# Autodesk Inventor assembly: B_Legs0_MIR
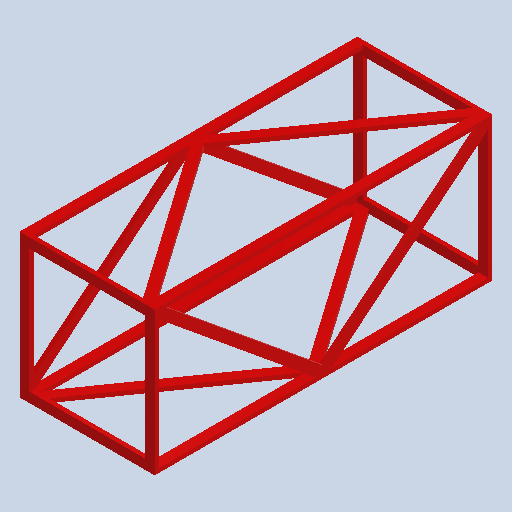
[picture p0: Inventor's stored thumbnail of the model, 512x512]
Saved by Autodesk Inventor 2025 (Build 290162000, 162)
## iProperties
Created: 2024-09-19
Part Number: B_Legs0_MIR
Document SubType Name: Assembly
Designer: localadmin
Author: User
## Documents named in this file (6)
- C:\Users\localadmin\Documents\USCTigerBurn24\Tburn24\F_Legs1\B_Legs0_MIR.iam
- C:\Users\localadmin\Documents\USCTigerBurn24\Tburn24\F_Legs1\8'x2x4_MIR.ipt
- C:\Users\localadmin\Documents\USCTigerBurn24\Tburn24\F_Legs1\4x2x4_MIR.ipt
- C:\Users\localadmin\Documents\USCTigerBurn24\Tburn24\F_Legs1\3'5x2x4_MIR.ipt
- C:\Users\localadmin\Documents\USCTigerBurn24\Tburn24\F_Legs1\side1_MIR.ipt
- C:\Users\localadmin\Documents\USCTigerBurn24\Tburn24\F_Legs1\side2_MIR.ipt
## Components (16 placed, 5 different names)
1. 8'x2x4_MIR:1 — Flush:3, Flush:2, Flush:1, Flush:14, Flush:13, Flush:8, Flush:12, Flush:10, Mate:3, Flush:22
2. 8'x2x4_MIR:2 — Flush:3, Flush:2, Flush:1, Mate:1, Flush:16, Flush:15, Mate:5, Flush:11, Flush:9, Flush:27, Flush:31, Mate:19, Flush:32, Mate:21
3. 4x2x4_MIR:1 — Flush:14, Flush:13, Flush:8, Mate:14, Flush:20, Flush:17, Mate:7, Flush:21, Mate:15, Flush:23, Mate:16, Flush:29
4. 4x2x4_MIR:2 — Flush:16, Flush:15, Mate:5, Flush:19, Flush:18, Mate:6, Mate:22
5. 4x2x4_MIR:3 — Flush:11, Flush:9, Flush:25, Flush:26
6. 4x2x4_MIR:4 — Flush:12, Flush:10, Mate:3, Mate:18, Mate:17
7. 8'x2x4_MIR:3 — Mate:14, Flush:20, Flush:17, Mate:7, Flush:24, Flush:30
8. 8'x2x4_MIR:4 — Flush:19, Flush:18, Mate:6, Flush:28
9. 3'5x2x4_MIR:1 — Flush:22, Flush:21, Mate:15
10. 3'5x2x4_MIR:2 — Flush:24, Flush:23, Mate:16
11. 3'5x2x4_MIR:3 — Flush:28, Flush:25, Mate:18
12. 3'5x2x4_MIR:4 — Flush:27, Flush:26, Mate:17, Mate:20
13. side1_MIR:1 — Flush:29
14. side2_MIR:1 — Flush:30
15. side2_MIR:2 — Flush:31, Mate:20, Mate:19
16. side1_MIR:2 — Flush:32, Mate:22, Mate:21
## Relationships (42: Flush 25, Mate 17)
- Flush:3: 8'x2x4_MIR:1 ↔ 8'x2x4_MIR:2
- Flush:2 (1130.3 mm): 8'x2x4_MIR:1 ↔ 8'x2x4_MIR:2
- Flush:1: 8'x2x4_MIR:1 ↔ 8'x2x4_MIR:2
- Mate:1: 8'x2x4_MIR:2
- Flush:14: 8'x2x4_MIR:1 ↔ 4x2x4_MIR:1
- Flush:13: 8'x2x4_MIR:1 ↔ 4x2x4_MIR:1
- Flush:8 [Mate]: 8'x2x4_MIR:1 ↔ 4x2x4_MIR:1
- Flush:16: 8'x2x4_MIR:2 ↔ 4x2x4_MIR:2
- Flush:15: 8'x2x4_MIR:2 ↔ 4x2x4_MIR:2
- Mate:5: 8'x2x4_MIR:2 ↔ 4x2x4_MIR:2
- Flush:11: 8'x2x4_MIR:2 ↔ 4x2x4_MIR:3
- Flush:9: 8'x2x4_MIR:2 ↔ 4x2x4_MIR:3
- Flush:12: 8'x2x4_MIR:1 ↔ 4x2x4_MIR:4
- Flush:10: 8'x2x4_MIR:1 ↔ 4x2x4_MIR:4
- Mate:3: 8'x2x4_MIR:1 ↔ 4x2x4_MIR:4
- Mate:14: 4x2x4_MIR:1 ↔ 8'x2x4_MIR:3
- Flush:20: 4x2x4_MIR:1 ↔ 8'x2x4_MIR:3
- Flush:17: 4x2x4_MIR:1 ↔ 8'x2x4_MIR:3
- Mate:7: 4x2x4_MIR:1 ↔ 8'x2x4_MIR:3
- Flush:19: 4x2x4_MIR:2 ↔ 8'x2x4_MIR:4
- Flush:18: 4x2x4_MIR:2 ↔ 8'x2x4_MIR:4
- Mate:6: 4x2x4_MIR:2 ↔ 8'x2x4_MIR:4
- Flush:22: 8'x2x4_MIR:1 ↔ 3'5x2x4_MIR:1
- Flush:21: 4x2x4_MIR:1 ↔ 3'5x2x4_MIR:1
- Mate:15: 4x2x4_MIR:1 ↔ 3'5x2x4_MIR:1
- Flush:24: 8'x2x4_MIR:3 ↔ 3'5x2x4_MIR:2
- Flush:23: 4x2x4_MIR:1 ↔ 3'5x2x4_MIR:2
- Mate:16: 4x2x4_MIR:1 ↔ 3'5x2x4_MIR:2
- Flush:28: 8'x2x4_MIR:4 ↔ 3'5x2x4_MIR:3
- Flush:25: 4x2x4_MIR:3 ↔ 3'5x2x4_MIR:3
- Mate:18: 4x2x4_MIR:4 ↔ 3'5x2x4_MIR:3
- Flush:27: 8'x2x4_MIR:2 ↔ 3'5x2x4_MIR:4
- Flush:26: 4x2x4_MIR:3 ↔ 3'5x2x4_MIR:4
- Mate:17: 4x2x4_MIR:4 ↔ 3'5x2x4_MIR:4
- Flush:29 [Mate]: 4x2x4_MIR:1 ↔ side1_MIR:1
- Flush:30 [Mate]: 8'x2x4_MIR:3 ↔ side2_MIR:1
- Flush:31: 8'x2x4_MIR:2 ↔ side2_MIR:2
- Mate:20: 3'5x2x4_MIR:4 ↔ side2_MIR:2
- Mate:19: 8'x2x4_MIR:2 ↔ side2_MIR:2
- Flush:32: 8'x2x4_MIR:2 ↔ side1_MIR:2
- Mate:22: 4x2x4_MIR:2 ↔ side1_MIR:2
- Mate:21: 8'x2x4_MIR:2 ↔ side1_MIR:2
